# Autodesk Inventor assembly: SistemaDeElevación
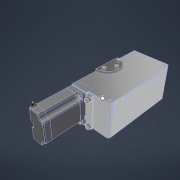
[picture p0: Inventor's stored thumbnail of the model, 180x180]
Saved by Autodesk Inventor 2022 (Build 260153000, 153)
## iProperties
Created: 2021-09-10
Part Number: SistemaDeElevación
Material: Generic
Document SubType Name: Assembly
Designer: Andres
Author: Andres
## Documents named in this file (19)
- D:\Documentos\15.PUCP_2021-2\[PDM] Proyecto de Diseño Mecatrónico\RobotPallet\SistemaDeElevación.iam
- D:\Documentos\15.PUCP_2021-2\[PDM] Proyecto de Diseño Mecatrónico\RobotPallet\Tornillo de elevación.ipt
- D:\Documentos\15.PUCP_2021-2\[PDM] Proyecto de Diseño Mecatrónico\RobotPallet\soporte de rodamientos.ipt
- D:\Documentos\15.PUCP_2021-2\[PDM] Proyecto de Diseño Mecatrónico\RobotPallet\SistemaDeElevación\Design Accelerator\Bevel Gears2.iam
- D:\Documentos\15.PUCP_2021-2\[PDM] Proyecto de Diseño Mecatrónico\RobotPallet\BridaTornillo.ipt
- D:\Documentos\15.PUCP_2021-2\[PDM] Proyecto de Diseño Mecatrónico\RobotPallet\NEMA 23 - 76mm.ipt
- D:\Documentos\15.PUCP_2021-2\[PDM] Proyecto de Diseño Mecatrónico\RobotPallet\Tuerca2.ipt
- D:\Documentos\15.PUCP_2021-2\[PDM] Proyecto de Diseño Mecatrónico\RobotPallet\SistemaDeElevación\Design Accelerator\Bearing3.iam
- D:\Documentos\15.PUCP_2021-2\[PDM] Proyecto de Diseño Mecatrónico\RobotPallet\Montura de Motor.ipt
- D:\Documentos\15.PUCP_2021-2\[PDM] Proyecto de Diseño Mecatrónico\RobotPallet\Cubierta.ipt
- D:\Documentos\15.PUCP_2021-2\[PDM] Proyecto de Diseño Mecatrónico\RobotPallet\ContentCenter\en-US\ISO 4762(2)\ISO 4762 - M3 x 12ISO.ipt
- D:\Documentos\15.PUCP_2021-2\[PDM] Proyecto de Diseño Mecatrónico\RobotPallet\ContentCenter\en-US\ISO 4762(2)\ISO 4762 - M5 x 16ISO.ipt
- D:\Documentos\15.PUCP_2021-2\[PDM] Proyecto de Diseño Mecatrónico\RobotPallet\ContentCenter\en-US\ISO 4762(2)\ISO 4762 - M4 x 12ISO.ipt
- D:\Documentos\15.PUCP_2021-2\[PDM] Proyecto de Diseño Mecatrónico\RobotPallet\ContentCenter\en-US\ISO 4762(2)\ISO 4762 - M4 x 10ISO.ipt
- D:\Documentos\15.PUCP_2021-2\[PDM] Proyecto de Diseño Mecatrónico\RobotPallet\ContentCenter\en-US\ISO 4762(2)\ISO 4762 - M4 x 6ISO.ipt
- D:\Documentos\15.PUCP_2021-2\[PDM] Proyecto de Diseño Mecatrónico\RobotPallet\SKF_KM 5.ipt
- D:\Documentos\15.PUCP_2021-2\[PDM] Proyecto de Diseño Mecatrónico\RobotPallet\SKF_MB 5.ipt
- D:\Documentos\15.PUCP_2021-2\[PDM] Proyecto de Diseño Mecatrónico\RobotPallet\AIS2021\SKF_7205 BE-2RZP.iam
- D:\Documentos\15.PUCP_2021-2\[PDM] Proyecto de Diseño Mecatrónico\RobotPallet\Brida de rodamientos.ipt
## Components (43 placed, 18 different names)
1. soporte de rodamientos:1 — Mate:8, Mate:17, Mate:18, Angle:2, Angle:3, Flush:1, Flush:2, Mate:19, Angle:4, Flush:3, Flush:4, Flush:5, Flush:6
2. Bevel Gears:1 [sub-assembly] — Mate:9, Mate:10, Mate:12, Mate:13, Mate:17, Mate:18, Angle:2
3. NEMA 23 - 76mm:1 — Mate:12, Angle:3, Insert:9, Insert:10, Insert:11, Insert:12
4. Tornillo de elevación:1 — Mate:3, Mate:6, Mate:16, Rigid:1, Angle:4, Rotation/Translation:1
5. BridaTornillo:1 — Mate:3, Elevación Tornillo, Mate:16, Rigid:1, Insert:19, Insert:20, Insert:21, Insert:22, Insert:23, Insert:24
6. Tuerca2:1 — Mate:6, Mate:8, Mate:9, Mate:10, Elevación Tornillo, Rigid:2, Rotation/Translation:1, Insert:13, Insert:14, Insert:15, Insert:16, Insert:17, Insert:18, Mate:20, Mate:21, Mate:22, Mate:25
7. Bearing:2 [sub-assembly] — Mate:13, Mate:19, Rigid:2
8. Montura de Motor:1 — Flush:1, Flush:2, Insert:5, Insert:6, Insert:7, Insert:8
9. Cubierta:1 — Flush:3, Flush:4, Insert:1, Insert:2, Insert:3, Insert:4
10. ISO 4762 M3 x 12:1 — Insert:1
11. ISO 4762 M3 x 12:2 — Insert:2
12. ISO 4762 M3 x 12:3 — Insert:3
13. ISO 4762 M3 x 12:4 — Insert:4
14. ISO 4762 M5 x 16:1 — Insert:5
15. ISO 4762 M5 x 16:2 — Insert:6
16. ISO 4762 M5 x 16:3 — Insert:7
17. ISO 4762 M5 x 16:4 — Insert:8
18. ISO 4762 M4 x 12:1 — Insert:9
19. ISO 4762 M4 x 12:2 — Insert:10
20. ISO 4762 M4 x 12:3 — Insert:11
21. ISO 4762 M4 x 12:4 — Insert:12
22. ISO 4762 M4 x 10:1 — Insert:13
23. ISO 4762 M4 x 10:2 — Insert:14
24. ISO 4762 M4 x 10:3 — Insert:15
25. ISO 4762 M4 x 10:4 — Insert:16
26. ISO 4762 M4 x 10:5 — Insert:17
27. ISO 4762 M4 x 10:6 — Insert:18
28. ISO 4762 M4 x 6:1 — Insert:19
29. ISO 4762 M4 x 6:2 — Insert:20
30. ISO 4762 M4 x 6:3 — Insert:21
31. ISO 4762 M4 x 6:4 — Insert:22
32. ISO 4762 M4 x 6:5 — Insert:23
33. ISO 4762 M4 x 6:6 — Insert:24
34. SKF_KM 5:1 — Mate:20, Mate:24
35. SKF_MB 5:1 — Mate:21, Mate:23, Mate:24
36. SKF_7205 BE-2RZP:1 [sub-assembly] — Mate:22, Mate:23, Mate:25
37. Brida de rodamientos:1 — Flush:5, Flush:6, Insert:25, Insert:26, Insert:27, Insert:28, Insert:29, Insert:30
38. ISO 4762 M4 x 10:7 — Insert:25
39. ISO 4762 M4 x 10:8 — Insert:26
40. ISO 4762 M4 x 10:9 — Insert:27
41. ISO 4762 M4 x 10:10 — Insert:28
42. ISO 4762 M4 x 10:11 — Insert:29
43. ISO 4762 M4 x 10:12 — Insert:30
## Relationships (60: Insert 30, Mate 18, Flush 6, Angle 3, WeldJoint 2, RelateRotateTranslate 1)
- Mate:3: Tornillo de elevación:1 ↔ BridaTornillo:1
- Mate:6: Tornillo de elevación:1 ↔ Tuerca2:1
- Mate:8: soporte de rodamientos:1 ↔ Tuerca2:1
- Mate:9: Bevel Gears:1 ↔ Tuerca2:1
- Mate:10: Bevel Gears:1 ↔ Tuerca2:1
- Elevación Tornillo [Mate]: BridaTornillo:1 ↔ Tuerca2:1
- Mate:12: Bevel Gears:1 ↔ NEMA 23 - 76mm:1
- Mate:13: Bevel Gears:1 ↔ Bearing:2
- Mate:16: Tornillo de elevación:1 ↔ BridaTornillo:1
- Rigid:1 [WeldJoint]: Tornillo de elevación:1 ↔ BridaTornillo:1
- Mate:17: soporte de rodamientos:1 ↔ Bevel Gears:1
- Mate:18: soporte de rodamientos:1 ↔ Bevel Gears:1
- Angle:2 (0 deg): soporte de rodamientos:1 ↔ Bevel Gears:1
- Angle:3 (0 deg): soporte de rodamientos:1 ↔ NEMA 23 - 76mm:1
- Flush:1: soporte de rodamientos:1 ↔ Montura de Motor:1
- Flush:2: soporte de rodamientos:1 ↔ Montura de Motor:1
- Mate:19: soporte de rodamientos:1 ↔ Bearing:2
- Rigid:2 [WeldJoint]: Tuerca2:1 ↔ Bearing:2
- Angle:4 (0 deg): soporte de rodamientos:1 ↔ Tornillo de elevación:1
- Rotation/Translation:1 [RelateRotateTranslate] (2 mm): Tornillo de elevación:1 ↔ Tuerca2:1
- Flush:3: soporte de rodamientos:1 ↔ Cubierta:1
- Flush:4: soporte de rodamientos:1 ↔ Cubierta:1
- Insert:1: Cubierta:1 ↔ ISO 4762 M3 x 12:1
- Insert:2: Cubierta:1 ↔ ISO 4762 M3 x 12:2
- Insert:3: Cubierta:1 ↔ ISO 4762 M3 x 12:3
- Insert:4: Cubierta:1 ↔ ISO 4762 M3 x 12:4
- Insert:5: Montura de Motor:1 ↔ ISO 4762 M5 x 16:1
- Insert:6: Montura de Motor:1 ↔ ISO 4762 M5 x 16:2
- Insert:7: Montura de Motor:1 ↔ ISO 4762 M5 x 16:3
- Insert:8: Montura de Motor:1 ↔ ISO 4762 M5 x 16:4
- Insert:9: NEMA 23 - 76mm:1 ↔ ISO 4762 M4 x 12:1
- Insert:10: NEMA 23 - 76mm:1 ↔ ISO 4762 M4 x 12:2
- Insert:11: NEMA 23 - 76mm:1 ↔ ISO 4762 M4 x 12:3
- Insert:12: NEMA 23 - 76mm:1 ↔ ISO 4762 M4 x 12:4
- Insert:13: Tuerca2:1 ↔ ISO 4762 M4 x 10:1
- Insert:14: Tuerca2:1 ↔ ISO 4762 M4 x 10:2
- Insert:15: Tuerca2:1 ↔ ISO 4762 M4 x 10:3
- Insert:16: Tuerca2:1 ↔ ISO 4762 M4 x 10:4
- Insert:17: Tuerca2:1 ↔ ISO 4762 M4 x 10:5
- Insert:18: Tuerca2:1 ↔ ISO 4762 M4 x 10:6
- Insert:19: BridaTornillo:1 ↔ ISO 4762 M4 x 6:1
- Insert:20: BridaTornillo:1 ↔ ISO 4762 M4 x 6:2
- Insert:21: BridaTornillo:1 ↔ ISO 4762 M4 x 6:3
- Insert:22: BridaTornillo:1 ↔ ISO 4762 M4 x 6:4
- Insert:23: BridaTornillo:1 ↔ ISO 4762 M4 x 6:5
- Insert:24: BridaTornillo:1 ↔ ISO 4762 M4 x 6:6
- Mate:20: Tuerca2:1 ↔ SKF_KM 5:1
- Mate:21: Tuerca2:1 ↔ SKF_MB 5:1
- Mate:22: Tuerca2:1 ↔ SKF_7205 BE-2RZP:1
- Mate:23: SKF_MB 5:1 ↔ SKF_7205 BE-2RZP:1
- Mate:24: SKF_KM 5:1 ↔ SKF_MB 5:1
- Mate:25: Tuerca2:1 ↔ SKF_7205 BE-2RZP:1
- Flush:5: soporte de rodamientos:1 ↔ Brida de rodamientos:1
- Flush:6: soporte de rodamientos:1 ↔ Brida de rodamientos:1
- Insert:25: Brida de rodamientos:1 ↔ ISO 4762 M4 x 10:7
- Insert:26: Brida de rodamientos:1 ↔ ISO 4762 M4 x 10:8
- Insert:27: Brida de rodamientos:1 ↔ ISO 4762 M4 x 10:9
- Insert:28: Brida de rodamientos:1 ↔ ISO 4762 M4 x 10:10
- Insert:29: Brida de rodamientos:1 ↔ ISO 4762 M4 x 10:11
- Insert:30: Brida de rodamientos:1 ↔ ISO 4762 M4 x 10:12
